# Autodesk Inventor assembly: VANT_ASSEMBLY
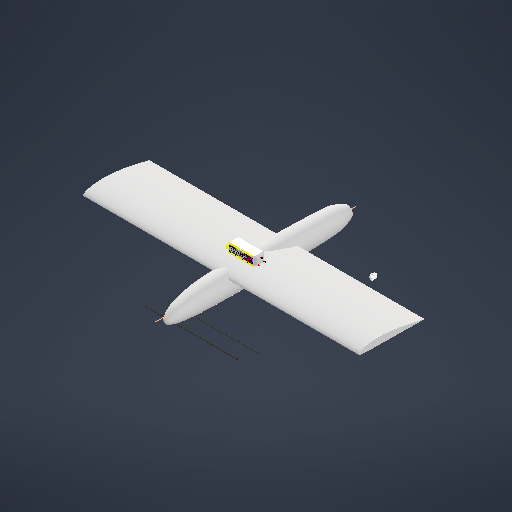
[picture p0: Inventor's stored thumbnail of the model, 512x512]
Saved by Autodesk Inventor 2026.1 (Build 301233000, 233)
## iProperties
Created: 2026-06-28
Part Number: VANT_ASSEMBLY
Document SubType Name: Assembly
Designer: adria
Author: adria
## Documents named in this file (9)
- C:\Users\adria\Desktop\VANT\VANT_ASSEMBLY.iam
- C:\Users\adria\Desktop\VANT\Airfoil.ipt
- C:\Users\adria\Desktop\VANT\Main_Body.ipt
- C:\Users\adria\Desktop\VANT\Hobbyocean EDF 70mm 12 blades.ipt
- C:\Users\adria\Desktop\VANT\Lipo Battery CNHL 4000mAh.ipt
- C:\Users\adria\Desktop\VANT\Assembly Micro Servo MG90S\Assembly Micro Servo MG90S\Assembly Micro Servo MG90S.iam
- C:\Users\adria\Desktop\VANT\Carbon Tube 8x6x500.ipt
- C:\Users\adria\Desktop\VANT\Carbon Tube 6x4x500.ipt
- C:\Users\adria\Downloads\abstract-dark-pattern\preview.jpg
## Components (8 placed, 7 different names)
1. Airfoil:1 — Flush:1, Mate:1, Angle:1
2. Main_Body:1 — Flush:2, Flush:3, Flush:4, Mate:1, Mate:2
3. Hobbyocean EDF 70mm 12 blades:1 — Flush:5, Mate:3
4. Lipo Battery CNHL 4000mAh:1 — Flush:6
5. Assembly Micro Servo MG90S:1 [sub-assembly]
6. Carbon Tube 8x6x500:1 — Flush:7
7. Carbon Tube 6x4x500:1 — Flush:8
8. Carbon Tube 6x4x500:2
## Relationships (12: Flush 8, Mate 3, Angle 1)
- Flush:1: Airfoil:1
- Flush:2: Main_Body:1
- Flush:3: Main_Body:1
- Flush:4: Main_Body:1
- Mate:1 (-330 mm): Airfoil:1 ↔ Main_Body:1
- Angle:1 (2 deg): Airfoil:1
- Flush:5: Hobbyocean EDF 70mm 12 blades:1
- Flush:6: Lipo Battery CNHL 4000mAh:1
- Mate:2: Main_Body:1
- Mate:3: Hobbyocean EDF 70mm 12 blades:1
- Flush:7: Carbon Tube 8x6x500:1
- Flush:8: Carbon Tube 6x4x500:1
